# Autodesk Inventor assembly: 9 polig stecker 10 grad
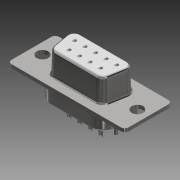
[picture p0: Inventor's stored thumbnail of the model, 180x180]
Saved by Autodesk Inventor 2017.3 (Build 213256000, 256)
## iProperties
Part Number: 9 polig stecker 10 grad
Material: Generisch
Document SubType Name: Assembly
Designer: Ljubko
Author: Ljubko
## Documents named in this file (5)
- C:\Users\Ljubko\Documents\Inventor\a steuerung\9 polig stecker.iam
- C:\Users\Ljubko\Documents\Inventor\a steuerung\9 polig o.ipt
- C:\Users\Ljubko\Documents\Inventor\a steuerung\9 polig u.ipt
- C:\Users\Ljubko\Documents\Inventor\a steuerung\kunst 9 polig.ipt
- C:\Users\Ljubko\Documents\Inventor\a steuerung\pin.ipt
## Components (12 placed, 4 different names)
1. 9 polig o:1 — Passend:1
2. 9 polig u:1 — Einfügen:1, Passend:10, Passend:11
3. kunst 9 polig:1 — Einfügen:1, Passend:1, Fluchtend:2
4. pin:1 — Fluchtend:13, Fluchtend:16
5. pin:2 — Fluchtend:12, Fluchtend:13, Fluchtend:15, Fluchtend:16
6. pin:3 — Fluchtend:11, Fluchtend:12, Fluchtend:14, Fluchtend:15
7. pin:4 — Fluchtend:11, Fluchtend:14, Fluchtend:19
8. pin:5 — Fluchtend:6, Fluchtend:19
9. pin:6 — Fluchtend:2, Fluchtend:3
10. pin:7 — Fluchtend:3, Fluchtend:4
11. pin:8 — Fluchtend:4, Fluchtend:5
12. pin:9 — Fluchtend:5, Fluchtend:6
## Relationships (16: Flush 12, Mate 3, Insert 1)
- Einfügen:1 [Insert]: 9 polig u:1 ↔ kunst 9 polig:1
- Passend:1 [Mate]: 9 polig o:1 ↔ kunst 9 polig:1
- Fluchtend:2 [Flush] (-3.3 mm): kunst 9 polig:1 ↔ pin:6
- Fluchtend:3 [Flush]: pin:6 ↔ pin:7
- Fluchtend:4 [Flush]: pin:7 ↔ pin:8
- Fluchtend:5 [Flush]: pin:8 ↔ pin:9
- Fluchtend:6 [Flush]: pin:5 ↔ pin:9
- Fluchtend:11 [Flush]: pin:3 ↔ pin:4
- Fluchtend:12 [Flush]: pin:2 ↔ pin:3
- Fluchtend:13 [Flush]: pin:1 ↔ pin:2
- Fluchtend:14 [Flush]: pin:3 ↔ pin:4
- Fluchtend:15 [Flush]: pin:2 ↔ pin:3
- Fluchtend:16 [Flush]: pin:1 ↔ pin:2
- Fluchtend:19 [Flush]: pin:4 ↔ pin:5
- Passend:10 [Mate]: 9 polig u:1
- Passend:11 [Mate]: 9 polig u:1
